# Autodesk Inventor assembly: wire_case-1
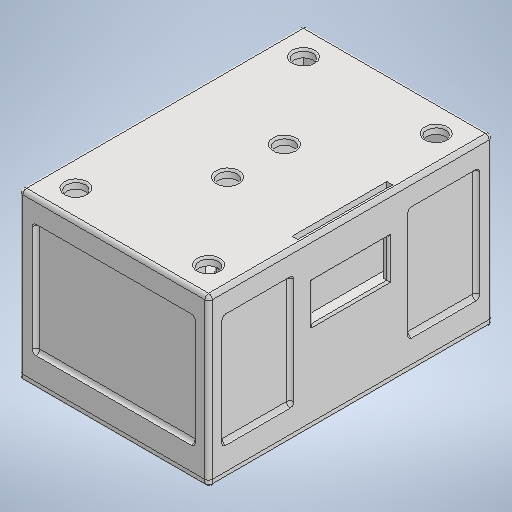
[picture p0: Inventor's stored thumbnail of the model, 512x512]
Saved by Autodesk Inventor 2025 (Build 290162000, 162)
## iProperties
Created: 2026-01-27
Part Number: wire_case-1
Document SubType Name: Assembly
Designer: mahhy
Author: mahhy
## Documents named in this file (7)
- C:\Users\mahhy\Documents\設計データ\wire_case-1\design-data\wire_case-1.iam
- C:\Users\mahhy\Documents\設計データ\wire_case-1\design-data\body-1.ipt
- C:\Users\mahhy\Documents\設計データ\wire_case-1\design-data\pole-1.ipt
- C:\Users\mahhy\Documents\設計データ\wire_case-1\design-data\body-2.ipt
- C:\Users\mahhy\Documents\設計データ\wire_case-1\design-data\box-1.ipt
- C:\Users\mahhy\Documents\設計データ\wire_case-1\design-data\box-2.ipt
- C:\Users\mahhy\Documents\設計データ\wire_case-1\design-data\cover-1.ipt
## Components (6 placed, 6 different names)
1. body-1:1 — メイト:1, メイト:2, メイト:3, メイト:4, メイト:5, メイト:6, メイト:10, メイト:11, メイト:12
2. pole-1:1 — 挿入:1
3. body-2:1 — 挿入:1, メイト:1, メイト:2, メイト:3
4. box-1:1 — メイト:4, メイト:5, メイト:6, メイト:7, メイト:9, メイト:8
5. box-2:1 — メイト:7, メイト:9, メイト:8
6. cover-1:1 — メイト:10, メイト:11, メイト:12
## Relationships (13: Mate 12, Insert 1)
- 挿入:1 [Insert]: pole-1:1 ↔ body-2:1
- メイト:1 [Mate]: body-1:1 ↔ body-2:1
- メイト:2 [Mate]: body-1:1 ↔ body-2:1
- メイト:3 [Mate]: body-1:1 ↔ body-2:1
- メイト:4 [Mate]: body-1:1 ↔ box-1:1
- メイト:5 [Mate]: body-1:1 ↔ box-1:1
- メイト:6 [Mate]: body-1:1 ↔ box-1:1
- メイト:7 [Mate]: box-1:1 ↔ box-2:1
- メイト:9 [Mate]: box-1:1 ↔ box-2:1
- メイト:8 [Mate]: box-1:1 ↔ box-2:1
- メイト:10 [Mate]: body-1:1 ↔ cover-1:1
- メイト:11 [Mate]: body-1:1 ↔ cover-1:1
- メイト:12 [Mate]: body-1:1 ↔ cover-1:1
